# Autodesk Inventor assembly: Bevel Drive Assembly
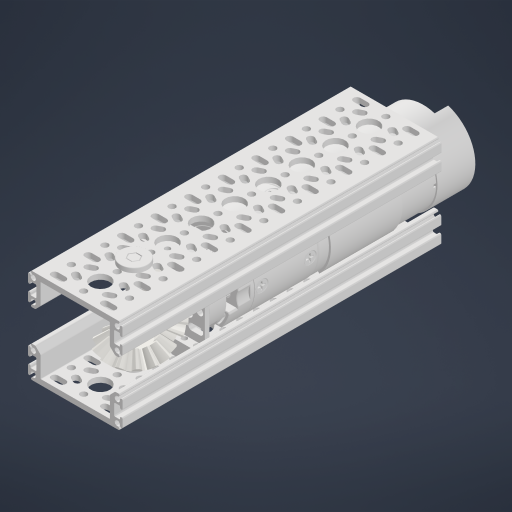
[picture p0: Inventor's stored thumbnail of the model, 512x512]
Saved by Autodesk Inventor 2023 (Build 270158000, 158)
## iProperties
Created: 2022-12-23
Part Number: Bevel Drive Assembly
Document SubType Name: Assembly
Designer: Izack Waczko
Author: Izack Waczko
## Documents named in this file (8)
- D:\CAD Modeling\Private Robotics\Custom Tryhard Robot\Drivetrain\Bevel Drive Assembly.iam
- D:\CAD Modeling\Private Robotics\Custom Tryhard Robot\Drivetrain\Bevel Drive\45mm x 15mm C Channel - 152mm.ipt
- D:\CAD Modeling\Private Robotics\Custom Tryhard Robot\Drivetrain\Bevel Drive\Rev C Channel Endcap.ipt
- D:\CAD Modeling\Private Robotics\Custom Tryhard Robot\Drivetrain\Bevel Drive\312rpm Gobilda Rex Motor.iam
- D:\CAD Modeling\Private Robotics\Custom Tryhard Robot\Drivetrain\Bevel Drive\1206-0016-0009.ipt
- D:\CAD Modeling\Private Robotics\Custom Tryhard Robot\Drivetrain\Bevel Drive\5mm x 55mm Hex Shaft.ipt
- D:\CAD Modeling\Private Robotics\Custom Tryhard Robot\Drivetrain\Bevel Drive\Through Bore Bearing Short.ipt
- D:\CAD Modeling\Private Robotics\Custom Tryhard Robot\Drivetrain\Bevel Drive Assembly\Design Accelerator\Bevel Gears1.iam
## Components (9 placed, 7 different names)
1. 45mm x 15mm C Channel - 152mm:1 — Mate:1, Mate:2, Mate:3, Mate:11, Mate:14
2. 45mm x 15mm C Channel - 152mm:2 — Mate:4, Mate:5, Mate:12, Mate:13
3. Rev C Channel Endcap:1 — Mate:1, Mate:2, Mate:3, Mate:4, Mate:5, Mate:6, Mate:7, Mate:8, Mate:17
4. 312rpm Gobilda Rex Motor:1 [sub-assembly] — Mate:9, Mate:10, Angle:1
5. 1206-0016-0009:1 — Mate:6, Mate:7, Mate:8, Mate:9, Mate:10
6. Through Bore Bearing Short:1 — Mate:11, Mate:14, Flush:1, Mate:15, Mate:16, Mate:18, Angle:2
7. Through Bore Bearing Short:2 — Mate:12, Mate:13
8. 5mm x 55mm Hex Shaft:1 — Flush:1, Mate:15, Mate:16
9. Bevel Gears:1 [sub-assembly] — Mate:17, Angle:1, Mate:18, Angle:2
## Relationships (21: Mate 18, Angle 2, Flush 1)
- Mate:1: 45mm x 15mm C Channel - 152mm:1 ↔ Rev C Channel Endcap:1
- Mate:2: 45mm x 15mm C Channel - 152mm:1 ↔ Rev C Channel Endcap:1
- Mate:3: 45mm x 15mm C Channel - 152mm:1 ↔ Rev C Channel Endcap:1
- Mate:4: 45mm x 15mm C Channel - 152mm:2 ↔ Rev C Channel Endcap:1
- Mate:5: 45mm x 15mm C Channel - 152mm:2 ↔ Rev C Channel Endcap:1
- Mate:6: Rev C Channel Endcap:1 ↔ 1206-0016-0009:1
- Mate:7: Rev C Channel Endcap:1 ↔ 1206-0016-0009:1
- Mate:8: Rev C Channel Endcap:1 ↔ 1206-0016-0009:1
- Mate:9: 312rpm Gobilda Rex Motor:1 ↔ 1206-0016-0009:1
- Mate:10: 312rpm Gobilda Rex Motor:1 ↔ 1206-0016-0009:1
- Mate:11: 45mm x 15mm C Channel - 152mm:1 ↔ Through Bore Bearing Short:1
- Mate:12: 45mm x 15mm C Channel - 152mm:2 ↔ Through Bore Bearing Short:2
- Mate:13: 45mm x 15mm C Channel - 152mm:2 ↔ Through Bore Bearing Short:2
- Mate:14: 45mm x 15mm C Channel - 152mm:1 ↔ Through Bore Bearing Short:1
- Flush:1: Through Bore Bearing Short:1 ↔ 5mm x 55mm Hex Shaft:1
- Mate:15: Through Bore Bearing Short:1 ↔ 5mm x 55mm Hex Shaft:1
- Mate:16: Through Bore Bearing Short:1 ↔ 5mm x 55mm Hex Shaft:1
- Mate:17: Rev C Channel Endcap:1 ↔ Bevel Gears:1
- Angle:1 (0 deg): 312rpm Gobilda Rex Motor:1 ↔ Bevel Gears:1
- Mate:18: Through Bore Bearing Short:1 ↔ Bevel Gears:1
- Angle:2 (0 deg): Through Bore Bearing Short:1 ↔ Bevel Gears:1
